# Autodesk Inventor assembly: Mark 6 - Frame
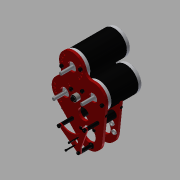
[picture p0: Inventor's stored thumbnail of the model, 180x180]
Saved by Autodesk Inventor 2013 (Build 170138000, 138)
## iProperties
Created: 2013-10-31
Part Number: Mark 6 - Frame
Document SubType Name: Assembly
Designer: grtstudent
Author: grtstudent
## Documents named in this file (25)
- C:\Users\grtstudent\Desktop\Mark 6 Final Preseason\Mark 6 - Frame.iam
- C:\Users\grtstudent\Desktop\Mark 6 Final Preseason\Plates\Mounting Plate\Mounting Plate Mark 7.ipt
- C:\Users\grtstudent\Desktop\Mark 6 Final Preseason\Plates\Mounting Plate\Main Connecting Standoff Thick.ipt
- C:\Users\grtstudent\Desktop\Mark 6 Final Preseason\Plates\Mounting Plate\Main Connecting Standoff Stepped.ipt
- C:\Users\grtstudent\Desktop\Mark 6 Final Preseason\Plates\Mounting Plate\.25-20 Pem Nut.ipt
- C:\Users\grtstudent\Desktop\Mark 6 Final Preseason\Plates\Mounting Plate\10-32 Flush Mounted Pem Nut.ipt
- C:\Users\grtstudent\Desktop\Mark 6 Final Preseason\Plates\Cim Plate\Cim Plate.ipt
- C:\Users\grtstudent\Desktop\Mark 6 Final Preseason\Plates\Pneumatic Plate\Pnuematic Plate.ipt
- C:\Users\grtstudent\Desktop\Mark 6 Final Preseason\Plates\Pneumatic Plate\Supporting Plate Standoff Thick.ipt
- C:\Users\grtstudent\Desktop\Mark 6 Final Preseason\Plates\Pneumatic Plate\4-40 Clinch Style Pem Nut .091 Minimum Panel Thickness.ipt
- C:\Users\grtstudent\Desktop\Mark 6 Final Preseason\Plates\Pneumatic Plate\Supporting Plate Standoff Thin.ipt
- C:\Users\grtstudent\Desktop\Mark 6 Final Preseason\Bolts\Socket Head Cap Screw 10-32 Thread 3.000 Length.ipt
- C:\Users\grtstudent\Desktop\Mark 6 Final Preseason\Bolts\Socket Head Cap Screw 10-32 Thread 2.500 Length.ipt
- C:\Users\grtstudent\Desktop\Mark 6 Final Preseason\Bolts\Button Head Cap Screw 8-32 Thread .250 Length.ipt
- C:\Users\grtstudent\Desktop\Mark 6 Final Preseason\Bolts\Socket Head Cap Screw 8-32 Thread 1.500 Length.ipt
- C:\Users\grtstudent\Desktop\Mark 6 Final Preseason\Bolts\Socket Head Cap Screw 4-40 Thread 1.125 Length.ipt
- C:\Users\grtstudent\Desktop\Mark 6 Final Preseason\Bolts\Socket Head Cap Screw 10-32 Thread .500 Length.ipt
- C:\Users\grtstudent\Desktop\Mark 6 Final Preseason\Bolts\Socket Head Cap Screw 6-32 Thread .500 Length.ipt
- C:\Users\grtstudent\Desktop\Mark 6 Final Preseason\Encoder\Encoder Mount.ipt
- C:\Users\grtstudent\Desktop\Mark 6 Final Preseason\Bolts\Button Head Cap Screw 6-32 Thread .250 Length.ipt
- C:\Users\grtstudent\Desktop\Mark 6 Final Preseason\Plates\Sheild.ipt
- C:\Users\grtstudent\Desktop\Mark 6 Final Preseason\Motors\CIM Can.ipt
- C:\Users\grtstudent\Desktop\Mark 6 Final Preseason\Motors\Mini CIM Can.ipt
- C:\Users\grtstudent\Desktop\Mark 6 Final Preseason\Motors\Rotor.ipt
- C:\Users\grtstudent\Desktop\Mark 6 Final Preseason\Bearings\R4-2RS.ipt
## Components (48 placed, 24 different names)
1. Cim Plate:1 — Mate:24, Mate:25, Mate:26, Mate:27, Mate:28, Mate:30, Mate:31, Mate:34, Mate:35, Mate:47, Mate:48, Mate:49, Mate:50, Mate:57, Mate:58, Mate:59, Mate:60, Mate:61, Mate:62, Mate:63, Mate:64, Mate:65, Mate:66, Mate:67, Mate:68, Mate:77, Mate:79, Mate:81, Mate:82, Mate:84, Mate:93, Mate:95, Mate:96
2. Encoder Mount:1 — Mate:73, Mate:74, Mate:75
3. Sheild:1 — Mate:84, Mate:85
4. R4-2RS:1 — Mate:101, Mate:102, Mate:103, Mate:104
5. R4-2RS:2 — Mate:101, Mate:102
6. Mounting Plate Mark 7:1 — Mate:1, Mate:2, Mate:3, Mate:4, Mate:5, Mate:6, Mate:7, Mate:8, Mate:9, Mate:10, Mate:11, Mate:12, Mate:13, Mate:14, Mate:15, Mate:16, Mate:17, Mate:18, Mate:19, Mate:20, Mate:21, Mate:22, Mate:23, Mate:69, Mate:70, Mate:71, Mate:72, Mate:73, Mate:74, Mate:75, Mate:76, Mate:78, Mate:80, Mate:83
7. Main Connecting Standoff Thick:1 — Mate:2, Mate:3, Mate:25, Mate:26
8. Main Connecting Standoff Thick:2 — Mate:1, Mate:4, Mate:24
9. Main Connecting Standoff Stepped:1 — Mate:5, Mate:6, Mate:45, Mate:46, Mate:103, Mate:104
10. .25-20 Pem Nut:1 — Mate:10, Mate:14
11. .25-20 Pem Nut:2 — Mate:9, Mate:13
12. .25-20 Pem Nut:3 — Mate:7, Mate:12
13. .25-20 Pem Nut:4 — Mate:8, Mate:11
14. 10-32 Flush Mounted Pem Nut:1 — Mate:15, Mate:18, Mate:22
15. 10-32 Flush Mounted Pem Nut:2 — Mate:17, Mate:20, Mate:21
16. 10-32 Flush Mounted Pem Nut:3 — Mate:16, Mate:19, Mate:23
17. Pnuematic Plate:1 — Mate:29, Mate:32, Mate:33, Mate:36, Mate:37, Mate:38, Mate:39, Mate:40, Mate:41, Mate:42, Mate:43, Mate:44, Mate:51, Mate:52, Mate:53, Mate:54, Mate:55, Mate:56
18. Supporting Plate Standoff Thick:1 — Mate:27, Mate:28, Mate:29
19. 4-40 Clinch Style Pem Nut .091 Minimum Panel Thickness:1 — Mate:37, Mate:40
20. Supporting Plate Standoff Thin:1 — Mate:30, Mate:32, Mate:35, Mate:36
21. 4-40 Clinch Style Pem Nut .091 Minimum Panel Thickness:2 — Mate:38, Mate:39
22. Supporting Plate Standoff Thin:2 — Mate:31, Mate:33, Mate:34
23. Socket Head Cap Screw 10-32 Thread 3.000 Length:1 — Mate:41, Mate:43
24. Socket Head Cap Screw 10-32 Thread 3.000 Length:2 — Mate:42, Mate:44
25. Socket Head Cap Screw 10-32 Thread 2.500 Length:1 — Mate:45, Mate:46
26. Button Head Cap Screw 8-32 Thread .250 Length:1 — Mate:47, Mate:50
27. Button Head Cap Screw 8-32 Thread .250 Length:2 — Mate:48, Mate:49
28. Socket Head Cap Screw 8-32 Thread 1.500 Length:1 — Mate:51, Mate:52
29. Socket Head Cap Screw 4-40 Thread 1.125 Length:1 — Mate:54, Mate:56
30. Socket Head Cap Screw 4-40 Thread 1.125 Length:2 — Mate:53, Mate:55
31. Socket Head Cap Screw 10-32 Thread .500 Length:1 — Mate:58, Mate:64, Mate:100
32. Socket Head Cap Screw 10-32 Thread .500 Length:2 — Mate:61, Mate:65, Mate:94
33. Socket Head Cap Screw 10-32 Thread .500 Length:3 — Mate:62, Mate:66, Mate:92
34. Socket Head Cap Screw 10-32 Thread .500 Length:4 — Mate:59, Mate:67, Mate:97
35. Socket Head Cap Screw 10-32 Thread .500 Length:5 — Mate:57, Mate:63, Mate:99
36. Socket Head Cap Screw 10-32 Thread .500 Length:6 — Mate:60, Mate:68, Mate:98
37. Socket Head Cap Screw 6-32 Thread .500 Length:1 — Mate:69, Mate:71
38. Socket Head Cap Screw 6-32 Thread .500 Length:2 — Mate:70, Mate:72
39. Button Head Cap Screw 6-32 Thread .250 Length:1 — Mate:76, Mate:83, Mate:85
40. Button Head Cap Screw 6-32 Thread .250 Length:2 — Mate:77, Mate:82
41. Button Head Cap Screw 6-32 Thread .250 Length:3 — Mate:78, Mate:80
42. Button Head Cap Screw 6-32 Thread .250 Length:4 — Mate:79, Mate:81
43. CIM Can:1 — Mate:89, Mate:90, Mate:92, Mate:93, Mate:94
44. CIM Can:2 — Mate:86, Mate:87, Mate:95, Mate:97, Mate:98
45. Mini CIM Can:1 — Mate:88, Mate:91, Mate:96, Mate:99, Mate:100
46. Rotor:2 — Mate:88, Mate:91
47. Rotor:3 — Mate:86, Mate:87
48. Rotor:4 — Mate:89, Mate:90
## Relationships (104: Mate 104)
- Mate:1: Mounting Plate Mark 7:1 ↔ Main Connecting Standoff Thick:2
- Mate:2: Mounting Plate Mark 7:1 ↔ Main Connecting Standoff Thick:1
- Mate:3: Mounting Plate Mark 7:1 ↔ Main Connecting Standoff Thick:1
- Mate:4: Mounting Plate Mark 7:1 ↔ Main Connecting Standoff Thick:2
- Mate:5: Mounting Plate Mark 7:1 ↔ Main Connecting Standoff Stepped:1
- Mate:6: Mounting Plate Mark 7:1 ↔ Main Connecting Standoff Stepped:1
- Mate:7: Mounting Plate Mark 7:1 ↔ .25-20 Pem Nut:3
- Mate:8: Mounting Plate Mark 7:1 ↔ .25-20 Pem Nut:4
- Mate:9: Mounting Plate Mark 7:1 ↔ .25-20 Pem Nut:2
- Mate:10: Mounting Plate Mark 7:1 ↔ .25-20 Pem Nut:1
- Mate:11: Mounting Plate Mark 7:1 ↔ .25-20 Pem Nut:4
- Mate:12: Mounting Plate Mark 7:1 ↔ .25-20 Pem Nut:3
- Mate:13: Mounting Plate Mark 7:1 ↔ .25-20 Pem Nut:2
- Mate:14: Mounting Plate Mark 7:1 ↔ .25-20 Pem Nut:1
- Mate:15: Mounting Plate Mark 7:1 ↔ 10-32 Flush Mounted Pem Nut:1
- Mate:16: Mounting Plate Mark 7:1 ↔ 10-32 Flush Mounted Pem Nut:3
- Mate:17: Mounting Plate Mark 7:1 ↔ 10-32 Flush Mounted Pem Nut:2
- Mate:18: Mounting Plate Mark 7:1 ↔ 10-32 Flush Mounted Pem Nut:1
- Mate:19: Mounting Plate Mark 7:1 ↔ 10-32 Flush Mounted Pem Nut:3
- Mate:20: Mounting Plate Mark 7:1 ↔ 10-32 Flush Mounted Pem Nut:2
- Mate:21: Mounting Plate Mark 7:1 ↔ 10-32 Flush Mounted Pem Nut:2
- Mate:22: Mounting Plate Mark 7:1 ↔ 10-32 Flush Mounted Pem Nut:1
- Mate:23: Mounting Plate Mark 7:1 ↔ 10-32 Flush Mounted Pem Nut:3
- Mate:24: Cim Plate:1 ↔ Main Connecting Standoff Thick:2
- Mate:25: Cim Plate:1 ↔ Main Connecting Standoff Thick:1
- Mate:26: Cim Plate:1 ↔ Main Connecting Standoff Thick:1
- Mate:27: Cim Plate:1 ↔ Supporting Plate Standoff Thick:1
- Mate:28: Cim Plate:1 ↔ Supporting Plate Standoff Thick:1
- Mate:29: Pnuematic Plate:1 ↔ Supporting Plate Standoff Thick:1
- Mate:30: Cim Plate:1 ↔ Supporting Plate Standoff Thin:1
- Mate:31: Cim Plate:1 ↔ Supporting Plate Standoff Thin:2
- Mate:32: Pnuematic Plate:1 ↔ Supporting Plate Standoff Thin:1
- Mate:33: Pnuematic Plate:1 ↔ Supporting Plate Standoff Thin:2
- Mate:34: Cim Plate:1 ↔ Supporting Plate Standoff Thin:2
- Mate:35: Cim Plate:1 ↔ Supporting Plate Standoff Thin:1
- Mate:36: Pnuematic Plate:1 ↔ Supporting Plate Standoff Thin:1
- Mate:37: Pnuematic Plate:1 ↔ 4-40 Clinch Style Pem Nut .091 Minimum Panel Thickness:1
- Mate:38: Pnuematic Plate:1 ↔ 4-40 Clinch Style Pem Nut .091 Minimum Panel Thickness:2
- Mate:39: Pnuematic Plate:1 ↔ 4-40 Clinch Style Pem Nut .091 Minimum Panel Thickness:2
- Mate:40: Pnuematic Plate:1 ↔ 4-40 Clinch Style Pem Nut .091 Minimum Panel Thickness:1
- Mate:41: Pnuematic Plate:1 ↔ Socket Head Cap Screw 10-32 Thread 3.000 Length:1
- Mate:42: Pnuematic Plate:1 ↔ Socket Head Cap Screw 10-32 Thread 3.000 Length:2
- Mate:43: Pnuematic Plate:1 ↔ Socket Head Cap Screw 10-32 Thread 3.000 Length:1
- Mate:44: Pnuematic Plate:1 ↔ Socket Head Cap Screw 10-32 Thread 3.000 Length:2
- Mate:45: Main Connecting Standoff Stepped:1 ↔ Socket Head Cap Screw 10-32 Thread 2.500 Length:1
- Mate:46: Main Connecting Standoff Stepped:1 ↔ Socket Head Cap Screw 10-32 Thread 2.500 Length:1
- Mate:47: Cim Plate:1 ↔ Button Head Cap Screw 8-32 Thread .250 Length:1
- Mate:48: Cim Plate:1 ↔ Button Head Cap Screw 8-32 Thread .250 Length:2
- Mate:49: Cim Plate:1 ↔ Button Head Cap Screw 8-32 Thread .250 Length:2
- Mate:50: Cim Plate:1 ↔ Button Head Cap Screw 8-32 Thread .250 Length:1
- Mate:51: Pnuematic Plate:1 ↔ Socket Head Cap Screw 8-32 Thread 1.500 Length:1
- Mate:52: Pnuematic Plate:1 ↔ Socket Head Cap Screw 8-32 Thread 1.500 Length:1
- Mate:53: Pnuematic Plate:1 ↔ Socket Head Cap Screw 4-40 Thread 1.125 Length:2
- Mate:54: Pnuematic Plate:1 ↔ Socket Head Cap Screw 4-40 Thread 1.125 Length:1
- Mate:55 (20.701 mm): Pnuematic Plate:1 ↔ Socket Head Cap Screw 4-40 Thread 1.125 Length:2
- Mate:56 (20.701 mm): Pnuematic Plate:1 ↔ Socket Head Cap Screw 4-40 Thread 1.125 Length:1
- Mate:57: Cim Plate:1 ↔ Socket Head Cap Screw 10-32 Thread .500 Length:5
- Mate:58: Cim Plate:1 ↔ Socket Head Cap Screw 10-32 Thread .500 Length:1
- Mate:59: Cim Plate:1 ↔ Socket Head Cap Screw 10-32 Thread .500 Length:4
- Mate:60: Cim Plate:1 ↔ Socket Head Cap Screw 10-32 Thread .500 Length:6
- Mate:61: Cim Plate:1 ↔ Socket Head Cap Screw 10-32 Thread .500 Length:2
- Mate:62: Cim Plate:1 ↔ Socket Head Cap Screw 10-32 Thread .500 Length:3
- Mate:63: Cim Plate:1 ↔ Socket Head Cap Screw 10-32 Thread .500 Length:5
- Mate:64: Cim Plate:1 ↔ Socket Head Cap Screw 10-32 Thread .500 Length:1
- Mate:65: Cim Plate:1 ↔ Socket Head Cap Screw 10-32 Thread .500 Length:2
- Mate:66: Cim Plate:1 ↔ Socket Head Cap Screw 10-32 Thread .500 Length:3
- Mate:67: Cim Plate:1 ↔ Socket Head Cap Screw 10-32 Thread .500 Length:4
- Mate:68: Cim Plate:1 ↔ Socket Head Cap Screw 10-32 Thread .500 Length:6
- Mate:69: Mounting Plate Mark 7:1 ↔ Socket Head Cap Screw 6-32 Thread .500 Length:1
- Mate:70: Mounting Plate Mark 7:1 ↔ Socket Head Cap Screw 6-32 Thread .500 Length:2
- Mate:71 (6.35 mm): Mounting Plate Mark 7:1 ↔ Socket Head Cap Screw 6-32 Thread .500 Length:1
- Mate:72 (6.35 mm): Mounting Plate Mark 7:1 ↔ Socket Head Cap Screw 6-32 Thread .500 Length:2
- Mate:73: Encoder Mount:1 ↔ Mounting Plate Mark 7:1
- Mate:74: Encoder Mount:1 ↔ Mounting Plate Mark 7:1
- Mate:75: Encoder Mount:1 ↔ Mounting Plate Mark 7:1
- Mate:76: Mounting Plate Mark 7:1 ↔ Button Head Cap Screw 6-32 Thread .250 Length:1
- Mate:77: Cim Plate:1 ↔ Button Head Cap Screw 6-32 Thread .250 Length:2
- Mate:78: Mounting Plate Mark 7:1 ↔ Button Head Cap Screw 6-32 Thread .250 Length:3
- Mate:79: Cim Plate:1 ↔ Button Head Cap Screw 6-32 Thread .250 Length:4
- Mate:80 (0.7937 mm): Mounting Plate Mark 7:1 ↔ Button Head Cap Screw 6-32 Thread .250 Length:3
- Mate:81 (0.7937 mm): Cim Plate:1 ↔ Button Head Cap Screw 6-32 Thread .250 Length:4
- Mate:82 (0.7937 mm): Cim Plate:1 ↔ Button Head Cap Screw 6-32 Thread .250 Length:2
- Mate:83 (0.7937 mm): Mounting Plate Mark 7:1 ↔ Button Head Cap Screw 6-32 Thread .250 Length:1
- Mate:84: Cim Plate:1 ↔ Sheild:1
- Mate:85: Sheild:1 ↔ Button Head Cap Screw 6-32 Thread .250 Length:1
- Mate:86: CIM Can:2 ↔ Rotor:3
- Mate:87: CIM Can:2 ↔ Rotor:3
- Mate:88: Mini CIM Can:1 ↔ Rotor:2
- Mate:89: CIM Can:1 ↔ Rotor:4
- Mate:90: CIM Can:1 ↔ Rotor:4
- Mate:91: Mini CIM Can:1 ↔ Rotor:2
- Mate:92: Socket Head Cap Screw 10-32 Thread .500 Length:3 ↔ CIM Can:1
- Mate:93: Cim Plate:1 ↔ CIM Can:1
- Mate:94: Socket Head Cap Screw 10-32 Thread .500 Length:2 ↔ CIM Can:1
- Mate:95: Cim Plate:1 ↔ CIM Can:2
- Mate:96: Cim Plate:1 ↔ Mini CIM Can:1
- Mate:97: Socket Head Cap Screw 10-32 Thread .500 Length:4 ↔ CIM Can:2
- Mate:98: Socket Head Cap Screw 10-32 Thread .500 Length:6 ↔ CIM Can:2
- Mate:99: Socket Head Cap Screw 10-32 Thread .500 Length:5 ↔ Mini CIM Can:1
- Mate:100: Socket Head Cap Screw 10-32 Thread .500 Length:1 ↔ Mini CIM Can:1
- Mate:101: R4-2RS:1 ↔ R4-2RS:2
- Mate:102: R4-2RS:1 ↔ R4-2RS:2
- Mate:103: R4-2RS:1 ↔ Main Connecting Standoff Stepped:1
- Mate:104: R4-2RS:1 ↔ Main Connecting Standoff Stepped:1
